# Autodesk Inventor assembly: Jig_assembly
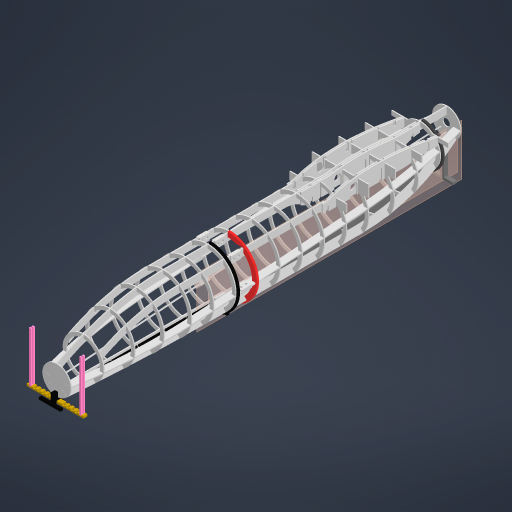
[picture p0: Inventor's stored thumbnail of the model, 512x512]
Saved by Autodesk Inventor 2023 (Build 270158000, 158)
## iProperties
Created: 2023-05-07
Part Number: Jig_assembly
Document SubType Name: Assembly
Designer: szykr
Author: szykr
## Documents named in this file (9)
- D:\Folder Instalacyjny\GitHub Pliki\Solaris\new model\Jig\Jig_assembly.iam
- D:\Folder Instalacyjny\GitHub Pliki\Solaris\new model\nowy kadłub.ipt
- D:\Folder Instalacyjny\GitHub Pliki\Solaris\new model\Jig\Jig_1.ipt
- D:\Folder Instalacyjny\GitHub Pliki\Solaris\new model\Jig\Front_aligner.ipt
- D:\Folder Instalacyjny\GitHub Pliki\Solaris\new model\Jig\Slider.ipt
- D:\Folder Instalacyjny\GitHub Pliki\Solaris\new model\Jig\Widełki.ipt
- D:\Folder Instalacyjny\GitHub Pliki\Solaris\new model\Jig\Jig_2.ipt
- D:\Folder Instalacyjny\GitHub Pliki\Solaris\new model\Jig\Back_front_aligner.ipt
- D:\Folder Instalacyjny\GitHub Pliki\Solaris\new model\Jig\Back_back_aligner.ipt
## Components (9 placed, 8 different names)
1. nowy kadłub:1 — Flush:2, Flush:6, Flush:7, Flush:8
2. Jig_1:1 — Flush:1, Flush:3
3. Front_aligner:1 — Flush:2
4. Slider:1 — Flush:3, Flush:4, Mate:1, Angle:1, Flush:5, Mate:2
5. Widełki:1 — Flush:4
6. Widełki:2 — Mate:1, Angle:1, Flush:5, Mate:2
7. Jig_2:1 — Flush:6
8. Back_front_aligner:1 — Flush:7
9. Back_back_aligner:1 — Flush:8
## Relationships (11: Flush 8, Mate 2, Angle 1)
- Flush:1: Jig_1:1
- Flush:2: nowy kadłub:1 ↔ Front_aligner:1
- Flush:3: Jig_1:1 ↔ Slider:1
- Flush:4: Slider:1 ↔ Widełki:1
- Mate:1 (0.1 mm): Slider:1 ↔ Widełki:2
- Angle:1 (180 deg): Slider:1 ↔ Widełki:2
- Flush:5 (0.1 mm): Slider:1 ↔ Widełki:2
- Mate:2 (0.1 mm): Slider:1 ↔ Widełki:2
- Flush:6: nowy kadłub:1 ↔ Jig_2:1
- Flush:7: nowy kadłub:1 ↔ Back_front_aligner:1
- Flush:8: nowy kadłub:1 ↔ Back_back_aligner:1
